# Autodesk Inventor assembly: lift
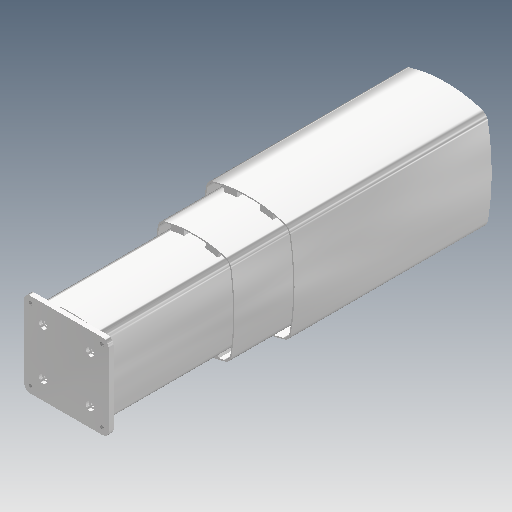
[picture p0: Inventor's stored thumbnail of the model, 512x512]
Saved by Autodesk Inventor 2020.3 (Build 243373000, 373)
## iProperties
Created: 2020-09-16
Part Number: lift
Document SubType Name: Assembly
Designer: Svend
Author: Svend
## Documents named in this file (5)
- C:\Users\Svend\OneDrive\Documents\GitHub\Rolstoel\lift.iam
- C:\Users\Svend\OneDrive\Documents\GitHub\Rolstoel\lineaire as deel 1.ipt
- C:\Users\Svend\OneDrive\Documents\GitHub\Rolstoel\lineaire as deel 2.ipt
- C:\Users\Svend\OneDrive\Documents\GitHub\Rolstoel\lineaire as deel 3.ipt
- C:\Users\Svend\OneDrive\Documents\GitHub\Rolstoel\plaat aan stoel.ipt
## Components (4 placed, 4 different names)
1. lineaire as deel 1:1 — Mate:1, Mate:3, Flush:1, Mate:6, Mate:7, Mate:8
2. lineaire as deel 2:1 — Mate:1, Mate:3, Flush:1, Mate:4, Mate:5, Flush:2
3. lineaire as deel 3:1 — Mate:4, Mate:5, Flush:2
4. plaat aan stoel:1 — Mate:6, Mate:7, Mate:8
## Relationships (9: Mate 7, Flush 2)
- Mate:1: lineaire as deel 1:1 ↔ lineaire as deel 2:1
- Mate:3: lineaire as deel 1:1 ↔ lineaire as deel 2:1
- Flush:1: lineaire as deel 1:1 ↔ lineaire as deel 2:1
- Mate:4: lineaire as deel 2:1 ↔ lineaire as deel 3:1
- Mate:5: lineaire as deel 2:1 ↔ lineaire as deel 3:1
- Flush:2: lineaire as deel 2:1 ↔ lineaire as deel 3:1
- Mate:6: lineaire as deel 1:1 ↔ plaat aan stoel:1
- Mate:7: lineaire as deel 1:1 ↔ plaat aan stoel:1
- Mate:8: lineaire as deel 1:1 ↔ plaat aan stoel:1
